# Autodesk Inventor assembly: motor_holder_assembly
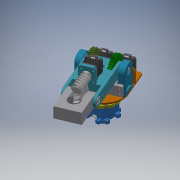
[picture p0: Inventor's stored thumbnail of the model, 180x180]
Saved by Autodesk Inventor 2019 (Build 230136000, 136)
## iProperties
Created: 2019-12-22
Part Number: motor_holder_assembly
Material: Типовые
Document SubType Name: Assembly
Designer: Петров Иван
Author: Петров Иван
## Documents named in this file (10)
- E:\IVAN\Ivan_desktop\Kvantorium\ROBOTS\Arm_manip\hardware\motor_holder_assembly.iam
- E:\IVAN\Ivan_desktop\Kvantorium\ROBOTS\Arm_manip\hardware\motor_holder.ipt
- E:\IVAN\Ivan_desktop\inventor\Models\Models\Motors and servo\motors\Stepper motors\nema-17-hs4401-s-1.snapshot.3\Nema 17HS4401-S.ipt
- E:\IVAN\Ivan_desktop\Kvantorium\ROBOTS\Arm_manip\hardware\gearbox_assembly.iam
- E:\IVAN\Ivan_desktop\Kvantorium\ROBOTS\Arm_manip\hardware\gearbox_secondary_gear_holder.ipt
- E:\IVAN\Ivan_desktop\Kvantorium\ROBOTS\Arm_manip\hardware\gearbox_main_gear.ipt
- E:\IVAN\Ivan_desktop\Kvantorium\ROBOTS\Arm_manip\hardware\gearbox_secondary_gear_as.ipt.iam
- E:\IVAN\Ivan_desktop\Kvantorium\ROBOTS\Arm_manip\hardware\gearbox_up.ipt
- E:\IVAN\Ivan_desktop\Kvantorium\ROBOTS\Arm_manip\hardware\joint_1_assembly.iam
- gearbox_secondary_gear_as.ipt
## Components (10 placed, 8 different names)
1. motor_holder:1 — Совмещение:1, Совмещение:2, Совмещение:3, Совмещение:4, Совмещение:6
2. Nema 17HS4401-S:1 — Совмещение:1, Совмещение:2, Совмещение:3, Совмещение:5, Совмещение:14, Совмещение:17
3. gearbox_assembly:1 [sub-assembly] — Совмещение:4, Совмещение:5, Совмещение:6, Совмещение:15, Совмещение:24, Совмещение:25
4. gearbox_secondary_gear_holder:1 — Совмещение:14, Совмещение:15, Совмещение:16, Совмещение:18, Совмещение:19, Совмещение:20, Совмещение:21, Совмещение:22, Совмещение:23
5. Цилиндрическое зубчатое зацепление2:1 — Совмещение:16, Совмещение:17
6. gearbox_secondary_gear_as.ipt:1 [sub-assembly] — Совмещение:18, Совмещение:19
7. gearbox_secondary_gear_as.ipt:2 [sub-assembly] — Совмещение:20, Совмещение:21
8. gearbox_secondary_gear_as.ipt:3 [sub-assembly] — Совмещение:22, Совмещение:23
9. gearbox_up:1 — Совмещение:24, Совмещение:25, Совмещение:26, Совмещение:27, Совмещение:28
10. joint_1_assembly:1 [sub-assembly] — Совмещение:26, Совмещение:27, Совмещение:28
## Relationships (21: Mate 21)
- Совмещение:1 [Mate]: motor_holder:1 ↔ Nema 17HS4401-S:1
- Совмещение:2 [Mate]: motor_holder:1 ↔ Nema 17HS4401-S:1
- Совмещение:3 [Mate]: motor_holder:1 ↔ Nema 17HS4401-S:1
- Совмещение:4 [Mate]: motor_holder:1 ↔ gearbox_assembly:1
- Совмещение:5 [Mate]: Nema 17HS4401-S:1 ↔ gearbox_assembly:1
- Совмещение:6 [Mate]: motor_holder:1 ↔ gearbox_assembly:1
- Совмещение:14 [Mate]: Nema 17HS4401-S:1 ↔ gearbox_secondary_gear_holder:1
- Совмещение:15 [Mate]: gearbox_assembly:1 ↔ gearbox_secondary_gear_holder:1
- Совмещение:16 [Mate]: gearbox_secondary_gear_holder:1 ↔ Цилиндрическое зубчатое зацепление2:1
- Совмещение:17 [Mate]: Nema 17HS4401-S:1 ↔ Цилиндрическое зубчатое зацепление2:1
- Совмещение:18 [Mate]: gearbox_secondary_gear_holder:1 ↔ gearbox_secondary_gear_as.ipt:1
- Совмещение:19 [Mate]: gearbox_secondary_gear_holder:1 ↔ gearbox_secondary_gear_as.ipt:1
- Совмещение:20 [Mate]: gearbox_secondary_gear_holder:1 ↔ gearbox_secondary_gear_as.ipt:2
- Совмещение:21 [Mate]: gearbox_secondary_gear_holder:1 ↔ gearbox_secondary_gear_as.ipt:2
- Совмещение:22 [Mate]: gearbox_secondary_gear_holder:1 ↔ gearbox_secondary_gear_as.ipt:3
- Совмещение:23 [Mate]: gearbox_secondary_gear_holder:1 ↔ gearbox_secondary_gear_as.ipt:3
- Совмещение:24 [Mate]: gearbox_assembly:1 ↔ gearbox_up:1
- Совмещение:25 [Mate]: gearbox_assembly:1 ↔ gearbox_up:1
- Совмещение:26 [Mate]: gearbox_up:1 ↔ joint_1_assembly:1
- Совмещение:27 [Mate]: gearbox_up:1 ↔ joint_1_assembly:1
- Совмещение:28 [Mate]: gearbox_up:1 ↔ joint_1_assembly:1
